# Autodesk Inventor assembly: GuideRail_MRS20
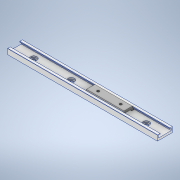
[picture p0: Inventor's stored thumbnail of the model, 180x180]
Saved by Autodesk Inventor 2022 (Build 260153000, 153)
## iProperties
Created: 2022-02-08
Part Number: GuideRail_MRS20
Document SubType Name: Assembly
Designer: satot
Author: satot
## Documents named in this file (3)
- C:\Users\satot\Documents\GrabCAD\NHK2022\BasicParts\SlideRail\GuideRail_MRS20\GuideRail_MRS20.iam
- C:\Users\satot\Documents\GrabCAD\NHK2022\BasicParts\SlideRail\GuideRail_MRS20\MRS20-200.ipt
- C:\Users\satot\Documents\GrabCAD\NHK2022\BasicParts\SlideRail\GuideRail_MRS20\MR-20CS.ipt
## Components (2 placed, 2 different names)
1. MRS20-200:1 — メイト:1, メイト:2
2. MR-20CS:1 — メイト:1, メイト:2
## Relationships (2: Mate 2)
- メイト:1 [Mate]: MRS20-200:1 ↔ MR-20CS:1
- メイト:2 [Mate]: MRS20-200:1 ↔ MR-20CS:1
